# Autodesk Inventor assembly: RobotPallet
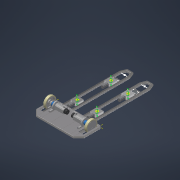
[picture p0: Inventor's stored thumbnail of the model, 180x180]
Saved by Autodesk Inventor 2022 (Build 260153000, 153)
## iProperties
Created: 2021-09-10
Part Number: RobotPallet
Material: Generic
Document SubType Name: Assembly
Designer: Andres
Author: Andres
## Documents named in this file (10)
- D:\Documentos\15.PUCP_2021-2\[PDM] Proyecto de Diseño Mecatrónico\ProyectoGIT\ProyectoRobotPallet\RobotPallet.iam
- D:\Documentos\15.PUCP_2021-2\[PDM] Proyecto de Diseño Mecatrónico\ProyectoGIT\ProyectoRobotPallet\Estructura Inferior\EstructuraInferior.iam
- D:\Documentos\15.PUCP_2021-2\[PDM] Proyecto de Diseño Mecatrónico\ProyectoGIT\ProyectoRobotPallet\Estructura Inferior\PlanchaBaseInferior.ipt
- D:\Documentos\15.PUCP_2021-2\[PDM] Proyecto de Diseño Mecatrónico\ProyectoGIT\ProyectoRobotPallet\Motor\BL Motor + Encoder + Gearbox + Rueda.iam
- D:\Documentos\15.PUCP_2021-2\[PDM] Proyecto de Diseño Mecatrónico\ProyectoGIT\ProyectoRobotPallet\ContentCenter\es-ES\DIN 630\DIN 630 - 2206 - 30 x 62 x 20.ipt
- D:\Documentos\15.PUCP_2021-2\[PDM] Proyecto de Diseño Mecatrónico\ProyectoGIT\ProyectoRobotPallet\Soportes\Soporte_Rodamiento.ipt
- D:\Documentos\15.PUCP_2021-2\[PDM] Proyecto de Diseño Mecatrónico\ProyectoGIT\ProyectoRobotPallet\Soportes\Soporte_Gearbox.ipt
- D:\Documentos\15.PUCP_2021-2\[PDM] Proyecto de Diseño Mecatrónico\ProyectoGIT\ProyectoRobotPallet\SistemaDeElevacion\version2\SistemaElevacionV2.iam
- SistemaElevacion2.iam
- D:\Documentos\15.PUCP_2021-2\[PDM] Proyecto de Diseño Mecatrónico\ProyectoGIT\ProyectoRobotPallet\RuedasAuxiliares\Ruedas de soporte.iam
## Components (16 placed, 8 different names)
1. EstructuraInferior:1 [sub-assembly] — Flush:1, Flush:13
2. PlanchaBaseInferior:1 — Flush:1
3. BL Motor + Encoder + Gearbox + Rueda:1 [sub-assembly] — Coincidencia:9, Nivelación:7, Coincidencia:19, Coincidencia:21, Mate:22
4. BL Motor + Encoder + Gearbox + Rueda:2 [sub-assembly] — Coincidencia:8, Nivelación:6, Coincidencia:16, Coincidencia:18, Mate:22
5. DIN 630 2206 - 30 x 62 x 20:1 — Coincidencia:8, Nivelación:6, Coincidencia:14, Nivelación:8
6. DIN 630 2206 - 30 x 62 x 20:2 — Coincidencia:9, Nivelación:7, Coincidencia:12, Nivelación:9
7. Soporte_Rodamiento:1 — Coincidencia:12, Nivelación:9
8. Soporte_Rodamiento:2 — Coincidencia:14, Nivelación:8
9. Soporte_Gearbox:1 — Coincidencia:16, Coincidencia:18
10. Soporte_Gearbox:2 — Coincidencia:19, Coincidencia:21
11. SistemaElevacion2:1 [sub-assembly] — Flush:11
12. SistemaElevacion2:2 [sub-assembly] — Flush:10, Flush:11
13. SistemaElevacion2:3 [sub-assembly] — Flush:10, Flush:12, Flush:13
14. SistemaElevacion2:4 [sub-assembly] — Flush:12
15. Ruedas de soporte:1 [sub-assembly] — Flush:14
16. Ruedas de soporte:2 [sub-assembly] — Flush:14
## Relationships (19: Flush 10, Mate 9)
- Flush:1: EstructuraInferior:1 ↔ PlanchaBaseInferior:1
- Coincidencia:8 [Mate]: BL Motor + Encoder + Gearbox + Rueda:2 ↔ DIN 630 2206 - 30 x 62 x 20:1
- Nivelación:6 [Flush] (-5 mm): BL Motor + Encoder + Gearbox + Rueda:2 ↔ DIN 630 2206 - 30 x 62 x 20:1
- Coincidencia:9 [Mate]: BL Motor + Encoder + Gearbox + Rueda:1 ↔ DIN 630 2206 - 30 x 62 x 20:2
- Nivelación:7 [Flush] (-5 mm): BL Motor + Encoder + Gearbox + Rueda:1 ↔ DIN 630 2206 - 30 x 62 x 20:2
- Coincidencia:12 [Mate]: DIN 630 2206 - 30 x 62 x 20:2 ↔ Soporte_Rodamiento:1
- Coincidencia:14 [Mate]: DIN 630 2206 - 30 x 62 x 20:1 ↔ Soporte_Rodamiento:2
- Nivelación:8 [Flush]: DIN 630 2206 - 30 x 62 x 20:1 ↔ Soporte_Rodamiento:2
- Nivelación:9 [Flush]: DIN 630 2206 - 30 x 62 x 20:2 ↔ Soporte_Rodamiento:1
- Coincidencia:16 [Mate]: BL Motor + Encoder + Gearbox + Rueda:2 ↔ Soporte_Gearbox:1
- Coincidencia:18 [Mate] (2.5 mm): BL Motor + Encoder + Gearbox + Rueda:2 ↔ Soporte_Gearbox:1
- Coincidencia:19 [Mate]: BL Motor + Encoder + Gearbox + Rueda:1 ↔ Soporte_Gearbox:2
- Coincidencia:21 [Mate] (2.5 mm): BL Motor + Encoder + Gearbox + Rueda:1 ↔ Soporte_Gearbox:2
- Mate:22: BL Motor + Encoder + Gearbox + Rueda:1 ↔ BL Motor + Encoder + Gearbox + Rueda:2
- Flush:10: SistemaElevacion2:2 ↔ SistemaElevacion2:3
- Flush:11: SistemaElevacion2:1 ↔ SistemaElevacion2:2
- Flush:12: SistemaElevacion2:3 ↔ SistemaElevacion2:4
- Flush:13: EstructuraInferior:1 ↔ SistemaElevacion2:3
- Flush:14: Ruedas de soporte:1 ↔ Ruedas de soporte:2
